# Autodesk Inventor assembly: tarot_5008_340kv_assy
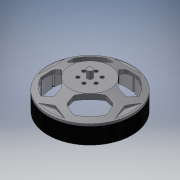
[picture p0: Inventor's stored thumbnail of the model, 180x180]
Saved by Autodesk Inventor 2019.4 (Build 234330000, 330)
## iProperties
Created: 2019-10-01
Part Number: tarot_5008_340kv_assy
Document SubType Name: Assembly
Designer: cdi
Author: cdi
## Documents named in this file (4)
- D:\SynologyDrive\workspace_inventor\2019_06_19.MT4008_actuator\tarot_5008_340kv\tarot_5008_340kv_assy.iam
- D:\SynologyDrive\workspace_inventor\2019_06_19.MT4008_actuator\tarot_5008_340kv\housing0.ipt
- D:\SynologyDrive\workspace_inventor\2019_06_19.MT4008_actuator\tarot_5008_340kv\housing1.ipt
- D:\SynologyDrive\workspace_inventor\2019_06_19.MT4008_actuator\tarot_5008_340kv\arc_magnet_10_10_2.ipt
## Components (16 placed, 3 different names)
1. housing0:1 — Mate:1, Mate:3, Mate:5
2. housing1:1 — Mate:2, Mate:3, Mate:6
3. arc_magnet_10_10_2:1 — Mate:5, Mate:6, Angle:1
4. arc_magnet_10_10_2:2
5. arc_magnet_10_10_2:3
6. arc_magnet_10_10_2:4
7. arc_magnet_10_10_2:5
8. arc_magnet_10_10_2:6
9. arc_magnet_10_10_2:7
10. arc_magnet_10_10_2:8
11. arc_magnet_10_10_2:9
12. arc_magnet_10_10_2:10
13. arc_magnet_10_10_2:11
14. arc_magnet_10_10_2:12
15. arc_magnet_10_10_2:13
16. arc_magnet_10_10_2:14
## Component patterns: (14 elements, first: arc_magnet_10_10_2:1)
## Relationships (6: Mate 5, Angle 1)
- Mate:1: housing0:1
- Mate:2: housing1:1
- Mate:3: housing0:1 ↔ housing1:1
- Mate:5: housing0:1 ↔ arc_magnet_10_10_2:1
- Mate:6: housing1:1 ↔ arc_magnet_10_10_2:1
- Angle:1 (0 deg): arc_magnet_10_10_2:1
